# Autodesk Inventor assembly: Assembly5
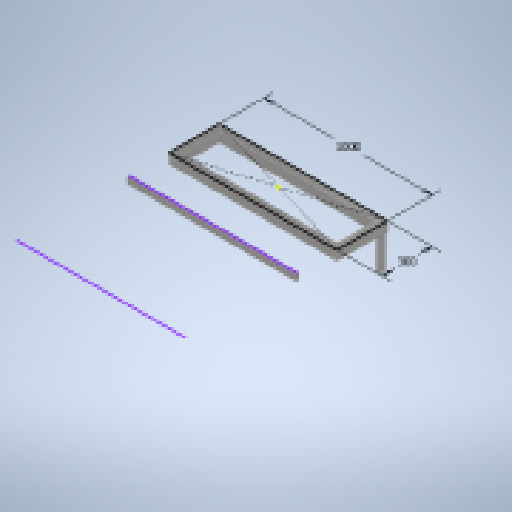
[picture p0: Inventor's stored thumbnail of the model, 512x512]
Saved by Autodesk Inventor 2025 (Build 290162010, 162A)
## iProperties
Created: 2024-08-28
Part Number: Assembly5
Document SubType Name: Assembly
Designer: admin
_SolveAssemblyDoc: Frame Generator Solve Assembly
_Version: 25.0.0
Author: admin
## Documents named in this file (4)
- C:\Users\admin\YandexDisk-badmisterfox\домашниий пк\Inventor\BSH_Beshkino_bio_tank\Assembly5.iam
- C:\Users\admin\YandexDisk-badmisterfox\домашниий пк\Inventor\BSH_Beshkino_bio_tank\Assembly5\Frame\Frame 1724863922149.iam
- C:\Users\admin\YandexDisk-badmisterfox\домашниий пк\Inventor\BSH_Beshkino_bio_tank\эскиз рамы.ipt
- C:\Users\admin\YandexDisk-badmisterfox\домашниий пк\Inventor\BSH_Beshkino_bio_tank\ISO 4019 - 40x20x2 - 0,001.ipt
## Components (4 placed, 3 different names)
1. эскиз рамы:1
2. Frame 1724863922149:1 [sub-assembly] — Rigid:1, Rigid:2
3. ISO 4019 - 40x20x2 - 0,001:1 — Rigid:1
4. ISO 4019 - 40x20x2 - 0,001:2 — Rigid:2
## Relationships (2: WeldJoint 2)
- Rigid:1 [WeldJoint]: Frame 1724863922149:1 ↔ ISO 4019 - 40x20x2 - 0,001:1
- Rigid:2 [WeldJoint]: Frame 1724863922149:1 ↔ ISO 4019 - 40x20x2 - 0,001:2
